# Autodesk Inventor assembly: Connessione-B
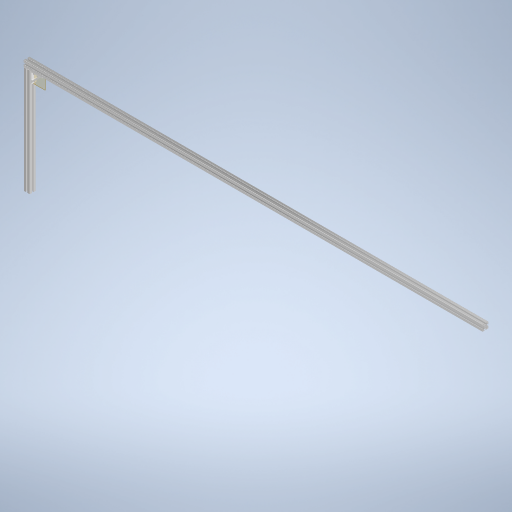
[picture p0: Inventor's stored thumbnail of the model, 512x512]
Saved by Autodesk Inventor 2023 (Build 270158000, 158)
## iProperties
Created: 2022-08-22
Part Number: Connessione-B
Document SubType Name: Assembly
Designer: matte
Author: matte
## Documents named in this file (6)
- C:\Users\matte\Documents\GitHub\MDM-CyberOrto-CAD\Dettagli\Connessione-B.iam
- C:\Users\matte\Documents\GitHub\MDM-CyberOrto-CAD\Pezzi singoli\Supporto SX.ipt
- C:\Users\matte\Documents\GitHub\MDM-CyberOrto-CAD\Parker components\03-Brackets_Gussets_Plates\09-Machined Gussets\20-102.ipt
- C:\Users\matte\Documents\GitHub\MDM-CyberOrto-CAD\Parker components\02-Fasteners\10-Standard T-Nuts\20-050.ipt
- C:\Users\matte\Documents\GitHub\MDM-CyberOrto-CAD\Parker components\02-Fasteners\16-Screws\01-Metric Screws\01-Button Head\24-118-8.ipt
- C:\Users\matte\Documents\GitHub\MDM-CyberOrto-CAD\Pezzi singoli\10-040.ipt
## Components (9 placed, 5 different names)
1. Supporto SX:1
2. 20-102:1
3. 20-050:1
4. 20-050:2
5. 24-118-8:1
6. 24-118-8:2
7. 24-118-8:3
8. 24-118-8:4
9. 10-040:1
## Relationships (20: Mate 17, Flush 3)
- [Mate]: 20-102:1 ↔ 10-040:1
- [Mate]: Supporto SX:1 ↔ 20-102:1
- [Flush]: Supporto SX:1 ↔ 20-102:1
- [Mate]: Supporto SX:1 ↔ 20-050:1
- [Mate]: 20-102:1 ↔ 20-050:1
- [Mate]: 20-102:1 ↔ 20-050:1
- [Mate]: 20-050:2 ↔ 10-040:1
- [Mate]: 20-102:1 ↔ 20-050:2
- [Mate]: 20-102:1 ↔ 20-050:2
- [Mate]: 20-102:1 ↔ 24-118-8:1
- [Mate]: 20-102:1 ↔ 24-118-8:1
- [Mate]: 20-102:1 ↔ 24-118-8:2
- [Mate]: 20-102:1 ↔ 24-118-8:2
- [Mate]: 20-102:1 ↔ 24-118-8:3
- [Mate]: 20-102:1 ↔ 24-118-8:3
- [Mate]: 20-102:1 ↔ 24-118-8:4
- [Mate]: 20-102:1 ↔ 24-118-8:4
- [Flush]: Supporto SX:1 ↔ 10-040:1
- [Mate]: Supporto SX:1 ↔ 10-040:1
- [Flush]: Supporto SX:1 ↔ 10-040:1
## Named parameters: d0_d9 = 0 mm, d1_d10 = 0 mm, d2_d11 = 0 mm, d3_d14 = 0 mm, d4_d15 = 0 mm, d5_d16 = 0 mm, d6_d17 = 0 mm, d7_d18 = 0 mm, d8_d19 = 0 mm
